# Autodesk Inventor assembly: Корпус 1 сборка
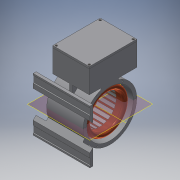
[picture p0: Inventor's stored thumbnail of the model, 180x180]
Saved by Autodesk Inventor 2016 SP1 (Build 200210100, 210)
## iProperties
Created: 2016-05-17
Part Number: Корпус 1 сборка
Material: Типовые
Document SubType Name: Assembly
Designer: a.kaluzhenin
Author: a.kaluzhenin
## Documents named in this file (7)
- H:\Projects\GitHub\mechatron\Корпус 1 сборка.iam
- H:\Projects\GitHub\mechatron\1 Корпус.ipt
- H:\Projects\GitHub\mechatron\Крышка контейнера.ipt
- H:\Projects\GitHub\mechatron\Сердечник корпуса.ipt
- H:\Projects\GitHub\mechatron\Вспомогательный цилиндр.ipt
- H:\Projects\GitHub\mechatron\Обмотка статора.ipt
- H:\Projects\GitHub\mechatron\Корпус 1 сборка\Мастер проектирования\Болтовое соединение1.iam
## Components (9 placed, 6 different names)
1. 1 Корпус:1 — Заподлицо:1, Совмещение:1, Заподлицо:2, Заподлицо:3, Заподлицо:4, Совмещение:5
2. Крышка контейнера:1 — Заподлицо:3, Заподлицо:4, Совмещение:5, Совмещение:6, Совмещение:7
3. Сердечник корпуса:1 — Заподлицо:5, Совмещение:3, Совмещение:4
4. Вспомогательный цилиндр:1 — Заподлицо:6, Угол:1
5. Обмотка статора:1 — Заподлицо:7
6. Болтовое соединение:1 [sub-assembly] — Совмещение:6, Совмещение:7
7. Болтовое соединение:2 [sub-assembly]
8. Болтовое соединение:3 [sub-assembly]
9. Болтовое соединение:4 [sub-assembly]
## Component patterns: (4 elements, first: Болтовое соединение:1)
## Relationships (14: Flush 7, Mate 6, Angle 1)
- Заподлицо:1 [Flush]: 1 Корпус:1
- Совмещение:1 [Mate]: 1 Корпус:1
- Заподлицо:2 [Flush]: 1 Корпус:1
- Заподлицо:3 [Flush]: 1 Корпус:1 ↔ Крышка контейнера:1
- Заподлицо:4 [Flush]: 1 Корпус:1 ↔ Крышка контейнера:1
- Заподлицо:5 [Flush]: Сердечник корпуса:1
- Заподлицо:6 [Flush]: Вспомогательный цилиндр:1
- Совмещение:3 [Mate]: Сердечник корпуса:1
- Угол:1 [Angle] (0 deg): Вспомогательный цилиндр:1
- Совмещение:4 [Mate]: Сердечник корпуса:1
- Заподлицо:7 [Flush]: Обмотка статора:1
- Совмещение:5 [Mate]: 1 Корпус:1 ↔ Крышка контейнера:1
- Совмещение:6 [Mate]: Крышка контейнера:1 ↔ Болтовое соединение:1
- Совмещение:7 [Mate]: Крышка контейнера:1 ↔ Болтовое соединение:1
